# Autodesk Inventor assembly: Eslabon_motor_R
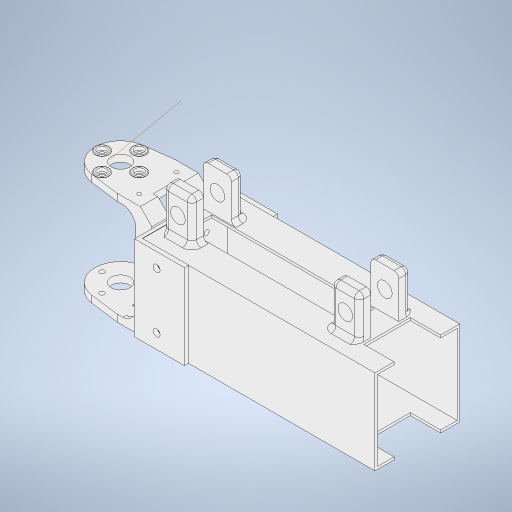
[picture p0: Inventor's stored thumbnail of the model, 512x512]
Saved by Autodesk Inventor 2024 (Build 280153000, 153)
## iProperties
Created: 2023-05-26
Part Number: Eslabon_motor_R
Document SubType Name: Assembly
Designer: epm01
Mass: 33.8172 g
Surface Area: 426.789 cm^2
Volume: 31.6279 cm^3
Author: epm01
## Documents named in this file (4)
- D:\Archivos\Inventor\Adaptable\Eslabon_motor_R.iam
- D:\Archivos\Inventor\Adaptable\Tapa_R.ipt
- D:\Archivos\Inventor\Adaptable\Eslabon_R.ipt
- D:\Archivos\Inventor\Adaptable\FP04-F2\FP04-F2.ipt
## Components (3 placed, 3 different names)
1. Tapa_R:1 — Coincidencia:1, Coincidencia:2, Coincidencia:3, Insertar:1
2. Eslabon_R:1 — Coincidencia:1, Coincidencia:2, Nivelación:1
3. FP04-F2:1 — Coincidencia:3, Insertar:1
## Relationships (5: Mate 3, Flush 1, Insert 1)
- Coincidencia:1 [Mate]: Tapa_R:1 ↔ Eslabon_R:1
- Coincidencia:2 [Mate]: Tapa_R:1 ↔ Eslabon_R:1
- Nivelación:1 [Flush] (-18.25 mm): Eslabon_R:1
- Coincidencia:3 [Mate]: Tapa_R:1 ↔ FP04-F2:1
- Insertar:1: Tapa_R:1 ↔ FP04-F2:1
